# Autodesk Inventor assembly: Pedal Assembly
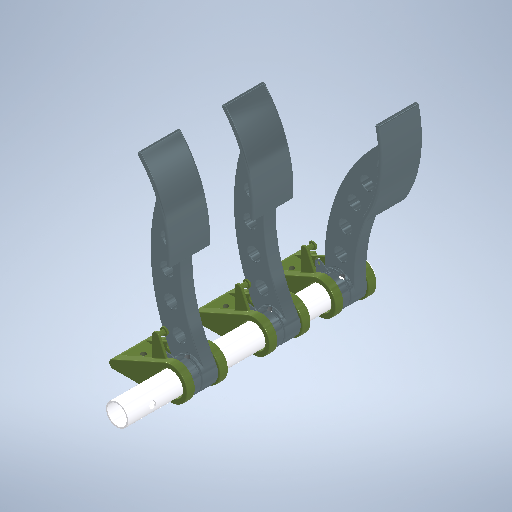
[picture p0: Inventor's stored thumbnail of the model, 512x512]
Saved by Autodesk Inventor 2025.2 (Build 292293000, 293)
## iProperties
Created: 2025-02-08
Part Number: Pedal Assembly
Document SubType Name: Assembly
Designer: eason
Author: eason
## Documents named in this file (4)
- C:\Users\eason\Desktop\Code\Unojoy-Simulator-Rig\CAD\Pedals\Pedal Assembly.iam
- C:\Users\eason\Desktop\Code\Unojoy-Simulator-Rig\CAD\Pedals\Steering PVC.ipt
- C:\Users\eason\Desktop\Code\Unojoy-Simulator-Rig\CAD\Pedals\Pedal Support.ipt
- C:\Users\eason\Desktop\Code\Unojoy-Simulator-Rig\CAD\Pedals\Pedal.ipt
## Components (7 placed, 3 different names)
1. Steering PVC:1 — Cylindrical:1, Cylindrical:2, Cylindrical:3, Cylindrical:4, Cylindrical:5, Cylindrical:6
2. Pedal Support:1 — Mate:1, Cylindrical:1, Mate:4, Mate:7
3. Pedal:1 — Cylindrical:4, Mate:4
4. Pedal Support:2 — Mate:2, Cylindrical:2, Mate:5, Mate:7, Mate:8
5. Pedal:2 — Cylindrical:5, Mate:5
6. Pedal Support:3 — Mate:3, Cylindrical:3, Mate:6, Mate:8
7. Pedal:3 — Cylindrical:6, Mate:6
## Relationships (14: Mate 8, CylindricalJoint 6)
- Mate:1: Pedal Support:1
- Mate:2: Pedal Support:2
- Mate:3: Pedal Support:3
- Cylindrical:1: Steering PVC:1 ↔ Pedal Support:1
- Cylindrical:2: Steering PVC:1 ↔ Pedal Support:2
- Cylindrical:3: Steering PVC:1 ↔ Pedal Support:3
- Cylindrical:4: Steering PVC:1 ↔ Pedal:1
- Mate:4: Pedal Support:1 ↔ Pedal:1
- Cylindrical:5: Steering PVC:1 ↔ Pedal:2
- Cylindrical:6: Steering PVC:1 ↔ Pedal:3
- Mate:5: Pedal Support:2 ↔ Pedal:2
- Mate:6: Pedal Support:3 ↔ Pedal:3
- Mate:7 (30 mm): Pedal Support:1 ↔ Pedal Support:2
- Mate:8 (50 mm): Pedal Support:2 ↔ Pedal Support:3
